# Autodesk Inventor assembly: Assembly1
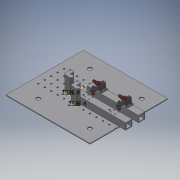
[picture p0: Inventor's stored thumbnail of the model, 180x180]
Saved by Autodesk Inventor 2018 (Build 220112000, 112)
## iProperties
Created: 2018-12-05
Part Number: Assembly1
Document SubType Name: Assembly
Designer: gbgic
Author: gbgic
## Documents named in this file (5)
- C:\Users\Gabriel\Documents\GitHub\2019CAD\Drill Jig Files\Drill Jig Assembly v1.iam
- C:\Users\Gabriel\Documents\GitHub\2019CAD\Drill Jig Files\Drill Jig Base.ipt
- C:\Users\Gabriel\Documents\GitHub\2019CAD\Drill Jig Files\Clamp Mount Aligner.ipt
- C:\Users\Gabriel\Documents\GitHub\2019CAD\Drill Jig Files\Toggle Clamp Files\305-U.iam
- C:\Users\Gabriel\Documents\GitHub\2019CAD\Drill Jig Files\Jig2.1_1x1_Bolt_Pattern_PIN.ipt
## Components (7 placed, 4 different names)
1. Drill Jig Base:1 — Mate:7, Mate:8, Mate:9, Mate:10, Mate:15, Mate:16, Mate:17, Mate:18
2. 305-U:1 [sub-assembly] — Mate:13
3. 305-U:2 [sub-assembly] — Mate:14
4. Jig2.1_1x1_Bolt_Pattern_PIN:1 — Mate:7, Mate:8
5. Jig2.1_1x1_Bolt_Pattern_PIN:2 — Mate:9, Mate:10
6. Clamp Mount Aligner:2 — Mate:13, Mate:14, Mate:15, Mate:16
7. Clamp Mount Aligner:3 — Mate:17, Mate:18
## Relationships (10: Mate 10)
- Mate:7: Drill Jig Base:1 ↔ Jig2.1_1x1_Bolt_Pattern_PIN:1
- Mate:8: Drill Jig Base:1 ↔ Jig2.1_1x1_Bolt_Pattern_PIN:1
- Mate:9: Drill Jig Base:1 ↔ Jig2.1_1x1_Bolt_Pattern_PIN:2
- Mate:10: Drill Jig Base:1 ↔ Jig2.1_1x1_Bolt_Pattern_PIN:2
- Mate:13: 305-U:1 ↔ Clamp Mount Aligner:2
- Mate:14: 305-U:2 ↔ Clamp Mount Aligner:2
- Mate:15: Drill Jig Base:1 ↔ Clamp Mount Aligner:2
- Mate:16: Drill Jig Base:1 ↔ Clamp Mount Aligner:2
- Mate:17: Drill Jig Base:1 ↔ Clamp Mount Aligner:3
- Mate:18: Drill Jig Base:1 ↔ Clamp Mount Aligner:3
